# Autodesk Inventor assembly: ASSEMBLED KEYBOARD
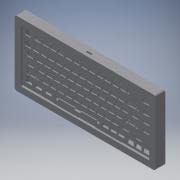
[picture p0: Inventor's stored thumbnail of the model, 180x180]
Saved by Autodesk Inventor 2017 (Build 210142000, 142)
## iProperties
Created: 2021-06-16
Part Number: ASSEMBLED KEYBOARD
Document SubType Name: Assembly
Designer: Jack
Author: Jack
## Documents named in this file (6)
- C:\Users\Jack\Desktop\custom keyboard\ASSEMBLED KEYBOARD.iam
- C:\Users\Jack\Desktop\custom keyboard\layer1.ipt
- C:\Users\Jack\Desktop\custom keyboard\layer2.ipt
- C:\Users\Jack\Desktop\custom keyboard\layer3.ipt
- C:\Users\Jack\Desktop\custom keyboard\layer4.ipt
- C:\Users\Jack\Desktop\custom keyboard\plate.ipt
## Components (7 placed, 5 different names)
1. layer1:1 — Mate:1, Rigid:1
2. layer2:1 — Mate:1, Rigid:1, Rigid:2
3. layer3:1 — Rigid:4, Rigid:5, Rigid:6
4. layer4:1 — Rigid:3, Rigid:4
5. plate:1 — Rigid:5
6. layer2:2 — Rigid:2, Rigid:3
7. layer2:3 — Rigid:6
## Relationships (7: WeldJoint 6, Mate 1)
- Mate:1: layer1:1 ↔ layer2:1
- Rigid:1 [WeldJoint]: layer1:1 ↔ layer2:1
- Rigid:2 [WeldJoint]: layer2:1 ↔ layer2:2
- Rigid:3 [WeldJoint]: layer4:1 ↔ layer2:2
- Rigid:4 [WeldJoint]: layer3:1 ↔ layer4:1
- Rigid:5 [WeldJoint] (-3 mm): layer3:1 ↔ plate:1
- Rigid:6 [WeldJoint]: layer3:1 ↔ layer2:3
